# Autodesk Inventor assembly: GE-12062
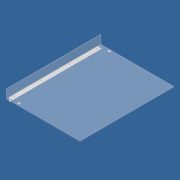
[picture p0: Inventor's stored thumbnail of the model, 180x180]
Saved by Autodesk Inventor 2012 (Build 160160000, 160)
## iProperties
Created: 2011-11-22
Part Number: GE-12062
Document SubType Name: Assembly
Designer: mcyr
Author: mcyr
## Documents named in this file (7)
- C:\Data Folder\FRC 2012 Field\Components\GE-12064.iam
- C:\Data Folder\FRC 2012 Field\Components\GE-12062.ipt
- C:\Data Folder\FRC 2012 Field\Components\GE-12063.ipt
- C:\Data Folder\FRC 2012 Field\Components\HW-00002.ipt
- C:\Data Folder\FRC 2012 Field\Components\HW-00012.ipt
- C:\Data Folder\FRC 2012 Field\Components\HW-00010.0002.ipt
- C:\Data Folder\FRC 2012 Field\Components\HW-00050.ipt
## Components (14 placed, 6 different names)
1. GE-12062:1 — Mate:1, Flush:1, Mate:2, Mate:3, Mate:4, Mate:7, Mate:8
2. GE-12063:1 — Mate:1, Flush:1, Mate:2, Mate:5
3. HW-00012:1 — Mate:3, Mate:4, Mate:6
4. HW-00002:1 — Mate:5, Mate:6
5. HW-00012:2
6. HW-00002:2
7. HW-00012:3
8. HW-00002:3
9. HW-00012:4
10. HW-00002:4
11. HW-00010.0002:1 — Mate:7, Mate:8, Mate:10, Mate:11
12. HW-00050:1 — Mate:10, Mate:11
13. HW-00010.0002:2
14. HW-00050:2
## Component patterns: (4 elements, first: HW-00012:1 + HW-00002:1), (2 elements, first: HW-00010.0002:1 + HW-00050:1)
## Relationships (11: Mate 10, Flush 1)
- Mate:1: GE-12062:1 ↔ GE-12063:1
- Flush:1: GE-12062:1 ↔ GE-12063:1
- Mate:2: GE-12062:1 ↔ GE-12063:1
- Mate:3: GE-12062:1 ↔ HW-00012:1
- Mate:4: GE-12062:1 ↔ HW-00012:1
- Mate:5: GE-12063:1 ↔ HW-00002:1
- Mate:6: HW-00012:1 ↔ HW-00002:1
- Mate:7: GE-12062:1 ↔ HW-00010.0002:1
- Mate:8 (3.175 mm): GE-12062:1 ↔ HW-00010.0002:1
- Mate:10: HW-00010.0002:1 ↔ HW-00050:1
- Mate:11: HW-00010.0002:1 ↔ HW-00050:1
